# Autodesk Inventor assembly: rotating_finger_B
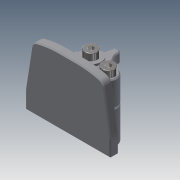
[picture p0: Inventor's stored thumbnail of the model, 180x180]
Saved by Autodesk Inventor 2018 (Build 220112000, 112)
## iProperties
Created: 2019-04-02
Part Number: rotating_finger_B
Document SubType Name: Assembly
Designer: Tsche
Author: Tsche
## Documents named in this file (6)
- C:\Users\Tsche\Documents\3d-printer\parts\grippers\Three_Finger_Gripper\BetaBots-Robot-Arm-Project-master\BetaBots-Robot-Arm-Project-master\ThreeFingerGripper\inventor\Gripper\cad_files\rotating_finger-tip\rotating_finger-tip_B.iam
- C:\Users\Tsche\Documents\3d-printer\parts\grippers\Three_Finger_Gripper\BetaBots-Robot-Arm-Project-master\BetaBots-Robot-Arm-Project-master\ThreeFingerGripper\inventor\Gripper\cad_files\rotating_finger-tip\rotating_finger-tip_finger-plain.ipt
- C:\Users\Tsche\Documents\3d-printer\parts\grippers\Three_Finger_Gripper\BetaBots-Robot-Arm-Project-master\BetaBots-Robot-Arm-Project-master\ThreeFingerGripper\inventor\Gripper\cad_files\rotating_finger-tip\rotating_finger-tip_spring-holder_B.ipt
- C:\Users\Tsche\Documents\3d-printer\parts\grippers\Three_Finger_Gripper\BetaBots-Robot-Arm-Project-master\BetaBots-Robot-Arm-Project-master\ThreeFingerGripper\inventor\Gripper\cad_files\rotating_finger-tip\rotating_finger-tip_bearing.ipt
- C:\Users\Tsche\Documents\3d-printer\parts\grippers\Three_Finger_Gripper\BetaBots-Robot-Arm-Project-master\BetaBots-Robot-Arm-Project-master\ThreeFingerGripper\inventor\Gripper\cad_files\rotating_finger-tip\rotating_finger-tip_limiter.ipt
- C:\Users\Tsche\Documents\3d-printer\parts\grippers\Three_Finger_Gripper\BetaBots-Robot-Arm-Project-master\BetaBots-Robot-Arm-Project-master\ThreeFingerGripper\inventor\Gripper\cad_files\rotating_finger-tip\Bolted Connection1.iam
## Components (7 placed, 5 different names)
1. rotating_finger-tip_finger-plain:1 — Mate:1, Mate:2, Mate:3, Mate:4, Cylindrical:1
2. rotating_finger-tip_bearing:1 — Mate:1, Mate:2, Flush:1
3. rotating_finger-tip_bearing:2 — Mate:3, Mate:4, Mate:10, Mate:11
4. rotating_finger-tip_spring-holder_B:1 — Flush:1, Cylindrical:1, Mate:5, Mate:6, Mate:7
5. rotating_finger-tip_limiter:1 — Mate:5, Mate:6, Mate:7, Mate:12, Mate:13
6. Bolted Connection:1 [sub-assembly] — Mate:12, Mate:13
7. Bolted Connection:2 [sub-assembly] — Mate:10, Mate:11
## Relationships (13: Mate 11, Flush 1, CylindricalJoint 1)
- Mate:1: rotating_finger-tip_finger-plain:1 ↔ rotating_finger-tip_bearing:1
- Mate:2: rotating_finger-tip_finger-plain:1 ↔ rotating_finger-tip_bearing:1
- Mate:3: rotating_finger-tip_finger-plain:1 ↔ rotating_finger-tip_bearing:2
- Mate:4: rotating_finger-tip_finger-plain:1 ↔ rotating_finger-tip_bearing:2
- Flush:1: rotating_finger-tip_bearing:1 ↔ rotating_finger-tip_spring-holder_B:1
- Cylindrical:1: rotating_finger-tip_finger-plain:1 ↔ rotating_finger-tip_spring-holder_B:1
- Mate:5: rotating_finger-tip_spring-holder_B:1 ↔ rotating_finger-tip_limiter:1
- Mate:6: rotating_finger-tip_spring-holder_B:1 ↔ rotating_finger-tip_limiter:1
- Mate:7: rotating_finger-tip_spring-holder_B:1 ↔ rotating_finger-tip_limiter:1
- Mate:10: rotating_finger-tip_bearing:2 ↔ Bolted Connection:2
- Mate:11: rotating_finger-tip_bearing:2 ↔ Bolted Connection:2
- Mate:12: rotating_finger-tip_limiter:1 ↔ Bolted Connection:1
- Mate:13: rotating_finger-tip_limiter:1 ↔ Bolted Connection:1
